# Autodesk Inventor assembly: Zonnepaneel V2.0
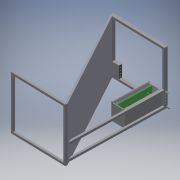
[picture p0: Inventor's stored thumbnail of the model, 180x180]
Saved by Autodesk Inventor 2018.3 (Build 223284000, 284)
## iProperties
Created: 2020-11-16
Part Number: Zonnepaneel V2.0
Document SubType Name: Assembly
Designer: daanv
Author: daanv
## Documents named in this file (7)
- C:\Users\daanv\OneDrive\Documenten\Life\Avans Project RED\Token\Zonnepaneel\V2.0\Zonnepaneel V2.0.iam
- C:\Users\daanv\OneDrive\Documenten\Life\Avans Project RED\Token\Zonnepaneel\V2.0\Zijplaat 1.ipt
- C:\Users\daanv\OneDrive\Documenten\Life\Avans Project RED\Token\Zonnepaneel\V2.0\Zijplaat 2.ipt
- C:\Users\daanv\OneDrive\Documenten\Life\Avans Project RED\Token\Zonnepaneel\V2.0\Zonnecel V2.0.ipt
- C:\Users\daanv\OneDrive\Documenten\Life\Avans Project RED\Token\Design 2\Token design 2.iam
- C:\Users\daanv\OneDrive\Documenten\Life\Avans Project RED\Token\Design 2\Pin Connector Curved.ipt
- C:\Users\daanv\OneDrive\Documenten\Life\Avans Project RED\Token\Design 2\4pin male and female.ipt
## Components (6 placed, 6 different names)
1. Zijplaat 1:1 — Mate:1, Mate:2, Mate:9, Mate:10, Mate:11, Mate:12, Mate:13, Mate:14
2. Zijplaat 2:1 — Mate:3, Mate:4, Mate:5
3. Zonnecel V2.0:1 — Mate:1, Mate:2, Mate:3, Mate:4, Mate:5
4. Token design 2:1 [sub-assembly] — Mate:6, Mate:7, Mate:8, Mate:9, Mate:10, Mate:11
5. Pin Connector Curved:1 — Mate:6, Mate:7, Mate:8
6. 4pin male and female:1 — Mate:12, Mate:13, Mate:14
## Relationships (14: Mate 14)
- Mate:1: Zijplaat 1:1 ↔ Zonnecel V2.0:1
- Mate:2: Zijplaat 1:1 ↔ Zonnecel V2.0:1
- Mate:3: Zijplaat 2:1 ↔ Zonnecel V2.0:1
- Mate:4: Zijplaat 2:1 ↔ Zonnecel V2.0:1
- Mate:5: Zijplaat 2:1 ↔ Zonnecel V2.0:1
- Mate:6: Token design 2:1 ↔ Pin Connector Curved:1
- Mate:7: Token design 2:1 ↔ Pin Connector Curved:1
- Mate:8: Token design 2:1 ↔ Pin Connector Curved:1
- Mate:9: Zijplaat 1:1 ↔ Token design 2:1
- Mate:10: Zijplaat 1:1 ↔ Token design 2:1
- Mate:11: Zijplaat 1:1 ↔ Token design 2:1
- Mate:12: Zijplaat 1:1 ↔ 4pin male and female:1
- Mate:13: Zijplaat 1:1 ↔ 4pin male and female:1
- Mate:14: Zijplaat 1:1 ↔ 4pin male and female:1
